# Autodesk Inventor assembly: Bearing Assembly
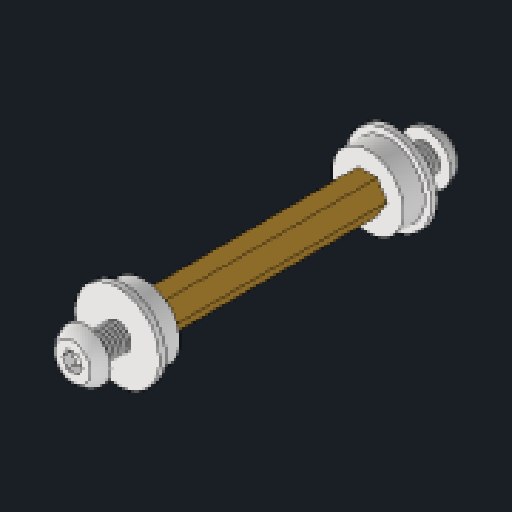
[picture p0: Inventor's stored thumbnail of the model, 512x512]
Saved by Autodesk Inventor 2023.2 (Build 272271030, 271C)
## iProperties
Created: 2024-02-28
Part Number: Bearing Assembly
Document SubType Name: Assembly
Designer: robpl
Author: robpl
## Documents named in this file (4)
- C:\Users\robpl\OneDrive\Documents\Arduino\Onslaught\CAD\Onslaught V2\Bearing Assembly.iam
- C:\Users\robpl\OneDrive\Documents\Arduino\Onslaught\CAD\Onslaught V2\M3 x 25mm Threaded Spacer.ipt
- C:\Users\robpl\OneDrive\Documents\Arduino\Onslaught\CAD\Onslaught V2\Bearing.ipt
- C:\Users\robpl\OneDrive\Documents\Arduino\Onslaught\CAD\Onslaught V2\M3 x 12 Button.ipt
## Components (5 placed, 3 different names)
1. M3 x 25mm Threaded Spacer:1 — Mate:1, Mate:2, Mate:3, Mate:4
2. Bearing:1 — Mate:1, Mate:4, Mate:5, Mate:6
3. Bearing:2 — Mate:2, Mate:3, Mate:7, Mate:8
4. M3 x 12 Button:1 — Mate:5, Mate:6
5. M3 x 12 Button:2 — Mate:7, Mate:8
## Relationships (8: Mate 8)
- Mate:1: M3 x 25mm Threaded Spacer:1 ↔ Bearing:1
- Mate:2: M3 x 25mm Threaded Spacer:1 ↔ Bearing:2
- Mate:3: M3 x 25mm Threaded Spacer:1 ↔ Bearing:2
- Mate:4: M3 x 25mm Threaded Spacer:1 ↔ Bearing:1
- Mate:5: Bearing:1 ↔ M3 x 12 Button:1
- Mate:6 (3.5 mm): Bearing:1 ↔ M3 x 12 Button:1
- Mate:7: Bearing:2 ↔ M3 x 12 Button:2
- Mate:8 (3.5 mm): Bearing:2 ↔ M3 x 12 Button:2
